# Autodesk Inventor assembly: Tail_Set
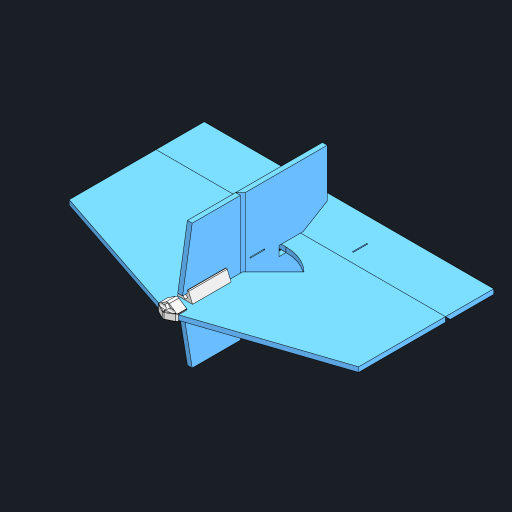
[picture p0: Inventor's stored thumbnail of the model, 512x512]
Saved by Autodesk Inventor 2023 (Build 270158000, 158)
## iProperties
Created: 2022-06-25
Part Number: Tail_Set
Document SubType Name: Assembly
Designer: legot
Author: legot
## Documents named in this file (7)
- C:\Users\legot\Documents\Inventor\HIKOSAPO\public_parts\Tail_Set.iam
- C:\Users\legot\Documents\Inventor\HIKOSAPO\OM\om_TailFrontHolder.ipt
- C:\Users\legot\Documents\Inventor\HIKOSAPO\OM\om_TailRod.ipt
- C:\Users\legot\Documents\Inventor\HIKOSAPO\public_parts\HoriMove.ipt
- C:\Users\legot\Documents\Inventor\HIKOSAPO\public_parts\HoriWing.ipt
- C:\Users\legot\Documents\Inventor\HIKOSAPO\public_parts\VertMove.ipt
- C:\Users\legot\Documents\Inventor\HIKOSAPO\public_parts\VertWing.ipt
## Components (6 placed, 6 different names)
1. om_TailFrontHolder:1 — フラッシュ:1, メイト:1, メイト:2, メイト:3, メイト:14, メイト:15
2. om_TailRod:1 — フラッシュ:1, メイト:1, メイト:8, メイト:9, メイト:10, メイト:16
3. HoriMove:1 — 角度:1, フラッシュ:3, メイト:13
4. HoriWing:1 — メイト:2, メイト:3, 角度:1, フラッシュ:3, メイト:13, メイト:14, メイト:15, メイト:16
5. VertMove:1 — メイト:11, フラッシュ:2, 角度:2
6. VertWing:1 — メイト:8, メイト:9, メイト:10, メイト:11, フラッシュ:2, 角度:2
## Relationships (16: Mate 11, Flush 3, Angle 2)
- フラッシュ:1 [Flush]: om_TailFrontHolder:1 ↔ om_TailRod:1
- メイト:1 [Mate]: om_TailFrontHolder:1 ↔ om_TailRod:1
- メイト:2 [Mate]: om_TailFrontHolder:1 ↔ HoriWing:1
- メイト:3 [Mate]: om_TailFrontHolder:1 ↔ HoriWing:1
- 角度:1 [Angle] (0 deg): HoriMove:1 ↔ HoriWing:1
- メイト:8 [Mate]: om_TailRod:1 ↔ VertWing:1
- メイト:9 [Mate]: om_TailRod:1 ↔ VertWing:1
- メイト:10 [Mate]: om_TailRod:1 ↔ VertWing:1
- メイト:11 [Mate]: VertMove:1 ↔ VertWing:1
- フラッシュ:2 [Flush]: VertMove:1 ↔ VertWing:1
- 角度:2 [Angle] (0 deg): VertMove:1 ↔ VertWing:1
- フラッシュ:3 [Flush]: HoriMove:1 ↔ HoriWing:1
- メイト:13 [Mate]: HoriMove:1 ↔ HoriWing:1
- メイト:14 [Mate]: om_TailFrontHolder:1 ↔ HoriWing:1
- メイト:15 [Mate]: om_TailFrontHolder:1 ↔ HoriWing:1
- メイト:16 [Mate]: om_TailRod:1 ↔ HoriWing:1
